# Autodesk Inventor assembly: 2parts_spool_motor
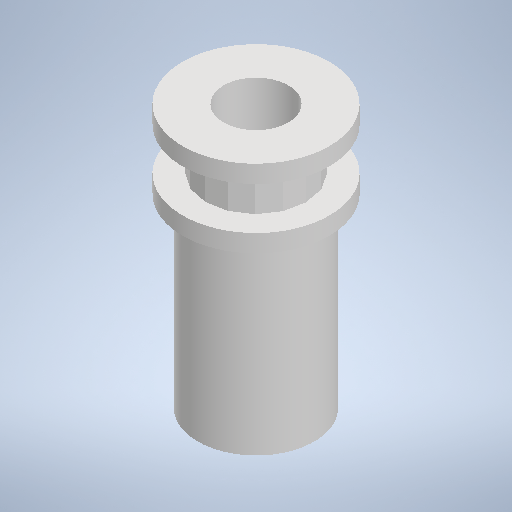
[picture p0: Inventor's stored thumbnail of the model, 512x512]
Saved by Autodesk Inventor 2025.2 (Build 292293000, 293)
## iProperties
Created: 2024-12-26
Part Number: 2parts_spool_motor
Document SubType Name: Assembly
Designer: Mos
Author: Mos
## Documents named in this file (3)
- C:\Users\Mos\Desktop\2parts_spool_motor.iam
- C:\Users\Mos\Desktop\spool_motor.ipt
- C:\Users\Mos\Desktop\spool_short.ipt
## Components (2 placed, 2 different names)
1. spool_motor:1 — Wstawiające:1
2. spool_short:1 — Wstawiające:1
## Relationships (1: Insert 1)
- Wstawiające:1 [Insert]: spool_motor:1 ↔ spool_short:1
